# Autodesk Inventor assembly: 098-DP(D-167)(F,D-166-1)
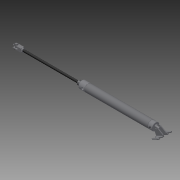
[picture p0: Inventor's stored thumbnail of the model, 180x180]
Saved by Autodesk Inventor 2014 (Build 180170000, 170)
## iProperties
Category: PARTsolutions
Company: BIMBA
Created: 2014-01-18
Part Number: 098-DP(D-167)(F,D-166-1)
Catalog Web Link: www.cadenas.de
Description: Original Line Standard Air Cylinders-
Vendor: BIMBA
Document SubType Name: Assembly
Designer: Andrew Toennies
Manufacturer: BIMBA
Mass: 77.5004 g
Surface Area: 709.854 cm^2
Volume: 77.5004 cm^3
Density: 1 g/cm^3
PSOL_IDENT_0: {$CADENAS_DATA\23d-libs\bimba\bimba\bimba_imperial\bimba_full_line\original_line_cylinders\standard_
PSOL_IDENT_1: air_cylinders\standard_air_cylinder_asmtab.prj},330 {VTYP=3D},{STYP=ASSTAB},{NB=098-DP(D-167)(F,D-16
PSOL_IDENT_2: 6-1)},{LINA=098-DP},{NN=Original Line Standard Air Cylinders},{DATE=11.10.2013 11:47:29},{GEOMDATE=1
PSOL_IDENT_3: 7.04.2013 07:27:53},{VERSION=},{LINEID=10},{LINESUBID=-1},{WBVAR=STROKE,ACTING,MNT,DER,NR,BM,CO,OO,V
PSOL_IDENT_4: O,M,EE,EEL,K,Q,Y,G,T,B,H,SER,SR,NT,W,HL,STPT1,STPT2,STPT3,STPT4,MB,PB,PRC,TB,MN}  {NB=098-DP(D-167)(
PSOL_IDENT_5: F,D-166-1)},{LINA=098-DP},{KT=DUMMY},{PN=098-DP},{PNC=098-DP(D-167)(F,D-166-1)},{PNA=(D-167)(D-166-1
PSOL_IDENT_6: )},{DASH=-},{BORE1=1.06250000},{BORE=1 1/16\" (09)},{BOREPN=09},{STROKE=8.000},{STROKEALG=[0.011:50/
PSOL_IDENT_7: 0.001]},{STROKE1=8.000},{ACTING=D},{ACTINGALG= '' , 'Single Acting (SA)' , 'R' , 'Reverse Single Act
PSOL_IDENT_8: ing (SA)' , 'D' , 'Double Acting (SA)' },{ACTINGPN=D},{MNT=P},{MNTALG= '' , 'Front Nose Mounting (SA
PSOL_IDENT_9: )' , 'P' , 'Rear Pivot Mounting (SA)' , 'X' , 'Universal Pivot Mounting or Double End Mounting (SA)'
PSOL_IDENT_10: , 'BF' , 'Front Block Mounting (SA)' , 'BR' , 'Rear Block Mounting for Vertical Positioning (SA)' ,
PSOL_IDENT_11: 'BFT' , 'Front Block Trunnion Mounting (SA)' , 'BRT' , 'Rear Block Trunnion Mounting (SA)' },{TYPE=
PSOL_IDENT_12: },{MNTPN=P},{DER=},{DERALG= '' , 'N/A' },{NR=},{NRALG= '' , 'N/A' },{NRPN=},{BM=},{BMALG= '' , 'N/A'
PSOL_IDENT_13: },{BMPN=},{CO=},{COALG= '' , 'N/A' },{OO=},{OOALG= '', 'N/A' },{OOPN=},{VO=Z},{VOALG= 'Z' , 'N/A' }
PSOL_IDENT_14: ,{VOPN=},{OOVOPN=},{M=},{MALG= '', 'Without Magnet', 'M', 'With Magnet' },{EE=},{EEL=0.000},{EEMAX=4
PSOL_IDENT_15: 2.0000},{EEALG= '', 'Without Extra Extension', 'EE', 'With Extra Extension' },{EELALG=0},{EEPN=},{EE
PSOL_IDENT_16: PN1=0.000},{K=},{KALG= '', 'Standard' , 'K' , 'Ports Rotated 90deg K' },{KPN=},{Q=},{QALG= '' , 'N/A'
PSOL_IDENT_17: },{QPN=},{Y=},{YALG= '' , 'Without Pivot Bushing' , 'Y' , 'With Pivot Bushing' },{YPN=},{YCON=},{F=
PSOL_IDENT_18: },{FALG= '', 'Non-Coated (Standard)', 'F', 'Molycoated' },{FPN=},{G=},{GPN=},{GPN99=},{T=},{TALG= ''
PSOL_IDENT_19: , 'Standard -20° to 200°F (-29° to 95°C)' , 'N' , 'Low Temperature' , 'V' , 'High Temperature' },{N
PSOL_IDENT_20: PN=},{VPN=},{B=},{BALG= '', 'W/out Bumpers' , 'B' , 'W/ Bumpers' },{BPN=},{H=},{HALG= '', 'N/A' },{H
PSOL_IDENT_21: PN=},{SER=},{SERALG= '' , 'Without Spring Extend/Return' , 'JS' , 'With Spring Return' , 'JR' , 'Wit
PSOL_IDENT_22: h Spring Extend' },{SR=C},{SRALG= 'C' , 'Standard Blackened Carbon Steel' , 'SR' , 'Stainless Steel
PSOL_IDENT_23: [SR]' },{SRPN=},{SRCON=1},{NT=},{NTPN=},{W=},{WALG= '' , 'Without Wiper' , 'W' , 'With Wiper' },{WPN=
PSOL_IDENT_24: },{E=},{EALG= '' , 'Standard Seals/Lube' , 'E' , 'Non-Lube Seals/Lube' },{EPN=},{HL=},{HLALG= '' , '
PSOL_IDENT_25: Without Low Pressure Hydraulic' , 'HL' , 'With Low Pressure Hydraulic' },{ST=},{STALG= '' , 'N/A' },
PSOL_IDENT_26: {STPT1=},{STPT1ALG= '' , 'N/A' },{STPT2=},{STPT2ALG= '' , 'N/A' },{STPT3=},{STPT3ALG= '' , 'N/A' },{
PSOL_IDENT_27: STPT4=},{STPT4ALG= '' , 'N/A' },{STPN=},{MB=},{MBALG= '' , 'N/A' },{MBPN=},{MBPNALL=},{MBPNALLREAR=}
PSOL_IDENT_28: ,{PB=D-167},{PBALG= '' , 'Without Pivot Bracket' , 'D-167' , 'D-167' },{PBPN=(D-167)},{PBPNALL=D-167
PSOL_IDENT_29: },{PRC=F,D-166-1},{PRCALG= '' , 'W/out Pivot Rod Clevis' , 'F,D-166-1' , 'D-166-1 (front)' },{PRCPN=
PSOL_IDENT_30: (F,D-166-1)},{PRCPNALL=D-166-1},{TB=},{TBALG= '' , 'N/A' },{TBPN=},{TBPNALL=},{MN=},{MNALG= '' , 'Wi
PSOL_IDENT_31: thout Mounting Nut' , 'F,D-9' , 'D-9 (front)'},{MNPN=},{MNCONF=},{MNCONR=},{TLEN=9.3185},{FRAC=74.84
PSOL_IDENT_32: 00},{RGCON=},{RGDACCON=R},{RHCON=P},{RHCON1=P},{RHCONON=1},{RHACCON=},{FNUTCON=0},{RNUTCON=0},{FNUTP
PSOL_IDENT_33: N=D-9},{RNUTPN=D-9},{FNUTTRANS=0.0000},{RNUTTRANS=0.0000},{VHOLECON=0},{A1=1.6250},{A1N=1.0000},{A1P=
PSOL_IDENT_34: 1.6250},{A1B=1.8750},{A4=0.2525},{A4N=0.3750},{A4P=0.2525},{A5=0.0300},{A1H=1.5},{A1NH=0.6250},{A1PH=
PSOL_IDENT_35: 1.5000},{A1BH=1.1250},{A1SH=1.1250},{A2H=0.2500},{A2NH=0.2500},{LENGTH=3.8400},{LENGTH1=3.8400},{LEN
PSOL_IDENT_36: GTH2=4.1000},{MUL=8.0000},{MUL11=8.0000},{MUL22=20.48},{MUL33=12.4800},{MUL2=8.0000},{MUL211=8.0000}
PSOL_IDENT_37: ,{MUL222=2.5600},{MUL233=1.5600},{SSS=16.0000},{RGLEN=1.4025},{RHLEN=0.9990},{SSS1=9.0000},{A13=1.21
PSOL_IDENT_38: 90},{DIF=0.1200},{G5=0.7180},{ON=0},{SSADD=0.0000},{BADD=0.0000},{MADD=0.0000},{NVADD=0.0000},{TRACK
PSOL_IDENT_39: L=9.0285},{TRACKCON=D-78527},{TRIMCON=0},{TRIMCON1=0},{PINCON=},{FSPACE=0.9348},{SPACE=0.1821},{TEXT=
PSOL_IDENT_40: 0.3188},{S1=1.2500},{D1=1.1410},{D1N=1.1130},{D1B=1.1130},{D1P=1.1410},{FA=0.940},{RA=0.9400},{PPATH=
PSOL_IDENT_41: standard_air_cylinder_asmtpl.prj},{MATALGHTML=<b>Standard Original Line:</b><dl><dt>Rod:</dt><dd>- S
PSOL_IDENT_42: tainless Steel</dd><dd>&nbsp;&nbsp;(5/16 9/16 Bores)</dd><dd>- High Strength Carbon Steel</dd><dd>&n
PSOL_IDENT_43: bsp;&nbsp;(3/4 3 Bore)</dd><dd>- Stainless Steel</dd><dd>&nbsp;&nbsp;(X style DXP/DX/DXDE)</dd><dt>B
PSOL_IDENT_44: earings:</dt><dd>- Sintered Bronze</dd><dt>Body:</dt><dd>- 304 Stainless Steel</dd><dt>End Caps:</dt
PSOL_IDENT_45: ><dd>- Aluminum</dd><dt>Seals:</dt><dd>- Buna N</dd></dl>},{ASSCFGPRA=09DP},{MBPNA=},{MNPNA=},{PRCPN
PSOL_IDENT_46: A=(D-166-1)},{ASSOPTACC=STPT4},{A=11.84},{HADD=0.0000},{WFL=0.125},{QADD=0.000},{QADD1=0.250},{TEST=
PSOL_IDENT_47: 8.0000},{MNTB=},{STDNUTF=0},{STDNUTR=0}
CNS_NN: Original Line Standard Air Cylinders
CNS_NT: Standard Male Thread
CNS_NB: 098-DP(D-167)(F,D-166-1)
CNS_NBSYN: $PNC.
CNS_LINA: 098-DP
CNS_PN: 098-DP
CNS_PNC: 098-DP(D-167)(F,D-166-1)
CNS_PNA: (D-167)(D-166-1)
CNS_DASH: -
CNS_BORE1: 1.06250000
CNS_BORE: 1 1/16" [09]
CNS_BOREPN: 09
CNS_STROKE: 8.000
CNS_STROKEALG: [0.011:50/0.001]
CNS_STROKE1: 8.000
CNS_ACTING: Double [D]
CNS_ACTINGALG: '' , 'Single Acting (SA)' , 'R' , 'Reverse Single Acting (SA)' , 'D' , 'Double Acting (SA)'
CNS_ACTINGPN: D
CNS_MNT: Rear Pivot [P]
CNS_MNTALG: '' , 'Front Nose Mounting (SA)' , 'P' , 'Rear Pivot Mounting (SA)' , 'X' , 'Universal Pivot Mounting or Double End Mounting (SA)' , 'BF' , 'Front Block Mounting (SA)' , 'BR' , 'Rear Block Mounting for Vertical Positioning (SA)' , 'BFT' , 'Front Block Trunnion Mounting (SA)' , 'BRT' , 'Rear Block Trunnion Mounting (SA)'
CNS_MNTPN: P
CNS_DER: N/A
CNS_DERALG: '' , 'N/A'
CNS_NR: N/A
CNS_NRALG: '' , 'N/A'
CNS_BM: N/A
CNS_BMALG: '' , 'N/A'
CNS_CO: N/A
CNS_COALG: '' , 'N/A'
CNS_OO: N/A
CNS_OOALG: '', 'N/A'
CNS_VO: N/A
CNS_VOALG: 'Z' , 'N/A'
CNS_M: Without Magnet Piston
CNS_MALG: '', 'Without Magnet', 'M', 'With Magnet'
CNS_EE: Standard Rod Extension
CNS_EEL: 0.000
CNS_EEMAX: 42.0000
CNS_EEALG: '', 'Without Extra Extension', 'EE', 'With Extra Extension'
CNS_EELALG: 0
CNS_EEPN1: 0.000
CNS_K: Standard
CNS_KALG: '', 'Standard' , 'K' , 'Ports Rotated 90deg K'
CNS_Q: N/A
CNS_QALG: '' , 'N/A'
CNS_Y: Standard Pivot Style
CNS_YALG: '' , 'Without Pivot Bushing' , 'Y' , 'With Pivot Bushing'
CNS_FALG: '', 'Non-Coated (Standard)', 'F', 'Molycoated'
CNS_G: Standard Grease Lube
CNS_T: Standard -20° to 200°F (-29° to 95°C)
CNS_TALG: '' , 'Standard -20° to 200°F (-29° to 95°C)' , 'N' , 'Low Temperature' , 'V' , 'High Temperature'
CNS_B: Without Bumpers
CNS_BALG: '', 'W/out Bumpers' , 'B' , 'W/ Bumpers'
CNS_H: N/A
CNS_HALG: '', 'N/A'
CNS_SER: Without Failsafe Spring Extend/Return
CNS_SERALG: '' , 'Without Spring Extend/Return' , 'JS' , 'With Spring Return' , 'JR' , 'With Spring Extend'
CNS_SR: Standard Blackened Carbon Steel
CNS_SRALG: 'C' , 'Standard Blackened Carbon Steel' , 'SR' , 'Stainless Steel [SR]'
CNS_SRCON: 1
CNS_W: Without Wiper
CNS_WALG: '' , 'Without Wiper' , 'W' , 'With Wiper'
CNS_EALG: '' , 'Standard Seals/Lube' , 'E' , 'Non-Lube Seals/Lube'
CNS_HL: Standard 250 PSI Air
CNS_HLALG: '' , 'Without Low Pressure Hydraulic' , 'HL' , 'With Low Pressure Hydraulic'
CNS_STALG: '' , 'N/A'
CNS_STPT1: N/A
CNS_STPT1ALG: '' , 'N/A'
CNS_STPT2: N/A
CNS_STPT2ALG: '' , 'N/A'
CNS_STPT3: N/A
CNS_STPT3ALG: '' , 'N/A'
CNS_STPT4: N/A
CNS_STPT4ALG: '' , 'N/A'
CNS_MB: N/A
CNS_MBALG: '' , 'N/A'
CNS_PB: D-167
CNS_PBALG: '' , 'Without Pivot Bracket' , 'D-167' , 'D-167'
CNS_PBPN: (D-167)
CNS_PBPNALL: D-167
CNS_PRC: D-166-1 (front)
CNS_PRCALG: '' , 'W/out Pivot Rod Clevis' , 'F,D-166-1' , 'D-166-1 (front)'
CNS_PRCPN: (F,D-166-1)
CNS_PRCPNALL: D-166-1
CNS_TB: N/A
CNS_TBALG: '' , 'N/A'
CNS_MN: Without Mounting Nut
CNS_MNALG: '' , 'Without Mounting Nut' , 'F,D-9' , 'D-9 (front)'
CNS_TLEN: 9.3185
CNS_FRAC: 74.8400
CNS_RGDACCON: R
CNS_RHCON: P
CNS_RHCON1: P
CNS_RHCONON: 1
CNS_FNUTCON: 0
CNS_RNUTCON: 0
CNS_FNUTPN: D-9
CNS_RNUTPN: D-9
CNS_FNUTTRANS: 0.0000
CNS_RNUTTRANS: 0.0000
CNS_VHOLECON: 0
CNS_A1: 1.6250
CNS_A1N: 1.0000
CNS_A1P: 1.6250
CNS_A1B: 1.8750
CNS_A4: 0.2525
CNS_A4N: 0.3750
CNS_A4P: 0.2525
CNS_A5: 0.0300
CNS_A1H: 1.500
CNS_A1NH: 0.6250
CNS_A1PH: 1.5000
CNS_A1BH: 1.1250
CNS_A1SH: 1.1250
CNS_A2H: 0.2500
CNS_A2NH: 0.2500
CNS_LENGTH: 3.8400
CNS_LENGTH1: 3.8400
CNS_LENGTH2: 4.1000
CNS_MUL: 8.0000
CNS_MUL11: 8.0000
CNS_MUL22: 20.480
CNS_MUL33: 12.4800
CNS_MUL2: 8.0000
CNS_MUL211: 8.0000
CNS_MUL222: 2.5600
CNS_MUL233: 1.5600
CNS_SSS: 16.0000
CNS_RGLEN: 1.4025
CNS_RHLEN: 0.9990
CNS_SSS1: 9.0000
CNS_A13: 1.2190
CNS_DIF: 0.1200
CNS_G5: 0.7180
CNS_ON: 0
CNS_SSADD: 0.0000
CNS_BADD: 0.0000
CNS_MADD: 0.0000
CNS_NVADD: 0.0000
CNS_TRACKL: 9.0285
CNS_TRACKCON: D-78527
CNS_TRIMCON: 0
CNS_TRIMCON1: 0
CNS_FSPACE: 0.9348
CNS_SPACE: 0.1821
CNS_TEXT: 0.3188
CNS_S1: 1.2500
CNS_D1: 1.1410
CNS_D1N: 1.1130
CNS_D1B: 1.1130
CNS_D1P: 1.1410
CNS_FA: 0.940
CNS_RA: 0.9400
CNS_PPATH: standard_air_cylinder_asmtpl.prj
CNS_MATALGHTML: <b>Standard Original Line:</b><dl><dt>Rod:</dt><dd>- Stainless Steel</dd><dd>&nbsp;&nbsp;(5/16 9/16 Bores)</dd><dd>- High Strength Carbon Steel</dd><dd>&nbsp;&nbsp;(3/4 3 Bore)</dd><dd>- Stainless Steel</dd><dd>&nbsp;&nbsp;(X style DXP/DX/DXDE)</dd><dt>Bearings:</dt><dd>- Sintered Bronze</dd><dt>Body:</dt><dd>- 304 Stainless Steel</dd><dt>End Caps:</dt><dd>- Aluminum</dd><dt>Seals:</dt><dd>- Buna N</dd></dl>
CNS_ASSCFGPRA: 09DP
CNS_PRCPNA: (D-166-1)
CNS_ASSOPTACC: STPT4
CNS_A: 11.84
CNS_HADD: 0.0000
CNS_WFL: 0.125
CNS_QADD: 0.000
CNS_QADD1: 0.250
CNS_TEST: 8.0000
CNS_STDNUTF: 0
CNS_STDNUTR: 0
SUPPLIER: BIMBA
ARTICLENO: 098-DP(D-167)(F,D-166-1)
BOMINFO: 098-DP
CREATOR: CADENAS GmbH
Title: 098-DP
Author: Cadenas PARTsolutions
## Documents named in this file (15)
- C:\Users\Andrew Toennies\Documents\GitHub\2014buildCAD\New Shooter\098-DP(D-167)(F,D-166-1).iam
- C:\Users\Andrew Toennies\Documents\GitHub\2014buildCAD\New Shooter\098-DPC(D-167)(F,D-166-1)0000_0_dummy.ipt
- C:\Users\Andrew Toennies\Documents\GitHub\2014buildCAD\New Shooter\09R000-0_rod_guide.ipt
- C:\Users\Andrew Toennies\Documents\GitHub\2014buildCAD\New Shooter\09R-9_31350C.ipt
- C:\Users\Andrew Toennies\Documents\GitHub\2014buildCAD\New Shooter\09P0000_rear_head.ipt
- C:\Users\Andrew Toennies\Documents\GitHub\2014buildCAD\New Shooter\D-51.ipt
- C:\Users\Andrew Toennies\Documents\GitHub\2014buildCAD\New Shooter\D-167-dummy.ipt
- C:\Users\Andrew Toennies\Documents\GitHub\2014buildCAD\New Shooter\D-168.ipt
- C:\Users\Andrew Toennies\Documents\GitHub\2014buildCAD\New Shooter\D-9966.ipt
- C:\Users\Andrew Toennies\Documents\GitHub\2014buildCAD\New Shooter\C-098-DP0_rod.ipt
- C:\Users\Andrew Toennies\Documents\GitHub\2014buildCAD\New Shooter\D-166-1-dummy.ipt
- C:\Users\Andrew Toennies\Documents\GitHub\2014buildCAD\New Shooter\D-14059.ipt
- C:\Users\Andrew Toennies\Documents\GitHub\2014buildCAD\New Shooter\D-8381.ipt
- C:\Users\Andrew Toennies\Documents\GitHub\2014buildCAD\New Shooter\D-5866.ipt
- C:\Users\Andrew Toennies\Documents\GitHub\2014buildCAD\New Shooter\D-746.ipt
## Components (15 placed, 14 different names)
1. 098-DPC(D-167)(F,D-166-1)0000_0_dummy:1 — dummy_XY@1 <-> rod_guide_XY@2, dummy_Z@1 <-> rod_guide_Z@2, dummy_YZ@1 <-> rod_guide_YZ@2
2. 09R000-0_rod_guide:1 — dummy_XY@1 <-> rod_guide_XY@2, dummy_Z@1 <-> rod_guide_Z@2, dummy_YZ@1 <-> rod_guide_YZ@2, to_tube_XY@2 <-> tube_front_XY@3, to_tube_Z@2 <-> tube_front_Z@3, to_tube_YZ@2 <-> tube_front_YZ@3, to_rod_XY@2 <-> rod_cp_XY@9, to_rod_Z@2 <-> rod_cp_Z@9
3. 09R-9_31350C:1 — to_tube_XY@2 <-> tube_front_XY@3, to_tube_Z@2 <-> tube_front_Z@3, to_tube_YZ@2 <-> tube_front_YZ@3, tube_rear_XY@3 <-> to_tube_XY@4, tube_rear_Z@3 <-> to_tube_Z@4, tube_rear_YZ@3 <-> to_tube_YZ@4
4. 09P0000_rear_head:1 — tube_rear_XY@3 <-> to_tube_XY@4, tube_rear_Z@3 <-> to_tube_Z@4, tube_rear_YZ@3 <-> to_tube_YZ@4, to_pin_XY@4 <-> pin_XY@5, to_pin_Z@4 <-> pin_Z@5, to_pin_YZ@4 <-> pin_YZ@5, to_pin_XY@4 <-> to_cyl_XY@6, to_pin_Z@4 <-> to_cyl_Z@6
5. D-51:1 — to_pin_XY@4 <-> pin_XY@5, to_pin_Z@4 <-> pin_Z@5, to_pin_YZ@4 <-> pin_YZ@5
6. D-167-dummy:1 — to_pin_XY@4 <-> to_cyl_XY@6, to_pin_Z@4 <-> to_cyl_Z@6, to_l_XY@6 <-> to_dummy_L_XY@7, to_l_Z@6 <-> to_dummy_L_Z@7, to_l_YZ@6 <-> to_dummy_L_YZ@7, to_r_XY@6 <-> to_dummy_R_XY@8, to_r_Z@6 <-> to_dummy_R_Z@8, to_r_YZ@6 <-> to_dummy_R_YZ@8
7. D-168:1 — to_l_XY@6 <-> to_dummy_L_XY@7, to_l_Z@6 <-> to_dummy_L_Z@7, to_l_YZ@6 <-> to_dummy_L_YZ@7
8. D-9966:1 — to_r_XY@6 <-> to_dummy_R_XY@8, to_r_Z@6 <-> to_dummy_R_Z@8, to_r_YZ@6 <-> to_dummy_R_YZ@8
9. C-098-DP0_rod:1 — to_rod_XY@2 <-> rod_cp_XY@9, to_rod_Z@2 <-> rod_cp_Z@9, to_rod_clevis_XY@9 <-> to_cyl_XY@10, to_rod_clevis_Z@9 <-> to_cyl_Z@10, to_rod_clevis_YZ@9 <-> to_cyl_YZ@10
10. D-166-1-dummy:1 — to_rod_clevis_XY@9 <-> to_cyl_XY@10, to_rod_clevis_Z@9 <-> to_cyl_Z@10, to_rod_clevis_YZ@9 <-> to_cyl_YZ@10, dummy_XY@10 <-> dummy_XY@11, dummy_Z@10 <-> dummy_Z@11, dummy_YZ@10 <-> dummy_YZ@11
11. D-14059:1 — dummy_XY@10 <-> dummy_XY@11, dummy_Z@10 <-> dummy_Z@11, dummy_YZ@10 <-> dummy_YZ@11, rod_clevis_body_XY@11 <-> pin_XY@12, rod_clevis_body_Z@11 <-> pin_Z@12, piston_rod_clevis_XY@11 <-> NUT_XY@15, piston_rod_clevis_Z@11 <-> NUT_Z@15
12. D-8381:1 — rod_clevis_body_XY@11 <-> pin_XY@12, rod_clevis_body_Z@11 <-> pin_Z@12, rr1_XY@12 <-> RR_XY@13, rr1_Z@12 <-> RR_Z@13, rr2_XY@12 <-> RR_XY@14, rr2_Z@12 <-> RR_Z@14
13. D-5866:1 — rr1_XY@12 <-> RR_XY@13, rr1_Z@12 <-> RR_Z@13
14. D-5866:2 — rr2_XY@12 <-> RR_XY@14, rr2_Z@12 <-> RR_Z@14
15. D-746:1 — piston_rod_clevis_XY@11 <-> NUT_XY@15, piston_rod_clevis_Z@11 <-> NUT_Z@15
## Relationships (36: Mate 20, Flush 8, Angle 8)
- dummy_XY@1 <-> rod_guide_XY@2 [Flush]: 098-DPC(D-167)(F,D-166-1)0000_0_dummy:1 ↔ 09R000-0_rod_guide:1
- dummy_Z@1 <-> rod_guide_Z@2 [Mate]: 098-DPC(D-167)(F,D-166-1)0000_0_dummy:1 ↔ 09R000-0_rod_guide:1
- dummy_YZ@1 <-> rod_guide_YZ@2 [Angle] (0 deg): 098-DPC(D-167)(F,D-166-1)0000_0_dummy:1 ↔ 09R000-0_rod_guide:1
- to_tube_XY@2 <-> tube_front_XY@3 [Flush]: 09R000-0_rod_guide:1 ↔ 09R-9_31350C:1
- to_tube_Z@2 <-> tube_front_Z@3 [Mate]: 09R000-0_rod_guide:1 ↔ 09R-9_31350C:1
- to_tube_YZ@2 <-> tube_front_YZ@3 [Angle] (0 deg): 09R000-0_rod_guide:1 ↔ 09R-9_31350C:1
- tube_rear_XY@3 <-> to_tube_XY@4 [Flush]: 09R-9_31350C:1 ↔ 09P0000_rear_head:1
- tube_rear_Z@3 <-> to_tube_Z@4 [Mate]: 09R-9_31350C:1 ↔ 09P0000_rear_head:1
- tube_rear_YZ@3 <-> to_tube_YZ@4 [Angle] (0 deg): 09R-9_31350C:1 ↔ 09P0000_rear_head:1
- to_pin_XY@4 <-> pin_XY@5 [Mate]: 09P0000_rear_head:1 ↔ D-51:1
- to_pin_Z@4 <-> pin_Z@5 [Mate]: 09P0000_rear_head:1 ↔ D-51:1
- to_pin_YZ@4 <-> pin_YZ@5 [Angle] (0 deg): 09P0000_rear_head:1 ↔ D-51:1
- to_pin_XY@4 <-> to_cyl_XY@6 [Flush]: 09P0000_rear_head:1 ↔ D-167-dummy:1
- to_pin_Z@4 <-> to_cyl_Z@6 [Mate]: 09P0000_rear_head:1 ↔ D-167-dummy:1
- to_l_XY@6 <-> to_dummy_L_XY@7 [Flush]: D-167-dummy:1 ↔ D-168:1
- to_l_Z@6 <-> to_dummy_L_Z@7 [Mate]: D-167-dummy:1 ↔ D-168:1
- to_l_YZ@6 <-> to_dummy_L_YZ@7 [Angle] (0 deg): D-167-dummy:1 ↔ D-168:1
- to_r_XY@6 <-> to_dummy_R_XY@8 [Flush]: D-167-dummy:1 ↔ D-9966:1
- to_r_Z@6 <-> to_dummy_R_Z@8 [Mate]: D-167-dummy:1 ↔ D-9966:1
- to_r_YZ@6 <-> to_dummy_R_YZ@8 [Angle] (0 deg): D-167-dummy:1 ↔ D-9966:1
- to_rod_XY@2 <-> rod_cp_XY@9 [Flush]: 09R000-0_rod_guide:1 ↔ C-098-DP0_rod:1
- to_rod_Z@2 <-> rod_cp_Z@9 [Mate]: 09R000-0_rod_guide:1 ↔ C-098-DP0_rod:1
- to_rod_clevis_XY@9 <-> to_cyl_XY@10 [Flush]: C-098-DP0_rod:1 ↔ D-166-1-dummy:1
- to_rod_clevis_Z@9 <-> to_cyl_Z@10 [Mate]: C-098-DP0_rod:1 ↔ D-166-1-dummy:1
- to_rod_clevis_YZ@9 <-> to_cyl_YZ@10 [Angle] (0 deg): C-098-DP0_rod:1 ↔ D-166-1-dummy:1
- dummy_XY@10 <-> dummy_XY@11 [Mate]: D-166-1-dummy:1 ↔ D-14059:1
- dummy_Z@10 <-> dummy_Z@11 [Mate]: D-166-1-dummy:1 ↔ D-14059:1
- dummy_YZ@10 <-> dummy_YZ@11 [Angle] (0 deg): D-166-1-dummy:1 ↔ D-14059:1
- rod_clevis_body_XY@11 <-> pin_XY@12 [Mate]: D-14059:1 ↔ D-8381:1
- rod_clevis_body_Z@11 <-> pin_Z@12 [Mate]: D-14059:1 ↔ D-8381:1
- rr1_XY@12 <-> RR_XY@13 [Mate]: D-8381:1 ↔ D-5866:1
- rr1_Z@12 <-> RR_Z@13 [Mate]: D-8381:1 ↔ D-5866:1
- rr2_XY@12 <-> RR_XY@14 [Mate]: D-8381:1 ↔ D-5866:2
- rr2_Z@12 <-> RR_Z@14 [Mate]: D-8381:1 ↔ D-5866:2
- piston_rod_clevis_XY@11 <-> NUT_XY@15 [Mate]: D-14059:1 ↔ D-746:1
- piston_rod_clevis_Z@11 <-> NUT_Z@15 [Mate]: D-14059:1 ↔ D-746:1
